# Autodesk Inventor assembly: Shrinkwrap Clamp
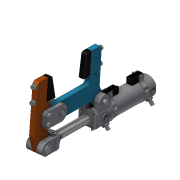
[picture p0: Inventor's stored thumbnail of the model, 180x180]
Saved by Autodesk Inventor 2020.1 (Build 241239000, 239)
## iProperties
Created: 2019-08-27
Part Number: Shrinkwrap Clamp
Document SubType Name: Assembly
Designer: thom_tremblay
Author: thom_tremblay
## Documents named in this file (5)
- C:\Users\thomastremblay\Desktop\Inventor ACP Data\Shrinkwrap Clamp.iam
- C:\Users\thomastremblay\Desktop\Inventor ACP Data\Assemblies\210-103c.iam
- C:\Users\thomastremblay\Desktop\Inventor ACP Data\Assemblies\210-110c.IAM
- C:\Users\thomastremblay\Desktop\Inventor ACP Data\Assemblies\PH-000-002.iam
- C:\Users\thomastremblay\Desktop\Inventor ACP Data\Assemblies\PH-000-001.iam
## Components (4 placed, 4 different names)
1. 210-103c:1 [sub-assembly]
2. 210-110c:1 [sub-assembly]
3. PH-000-002:1 [sub-assembly] — Insert:4
4. PH-000-001:1 [sub-assembly] — Insert:4
## Relationships (6: Insert 4, Mate 2)
- [Insert]: 210-103c:1 ↔ 210-110c:1
- [Insert]: 210-103c:1 ↔ PH-000-001:1
- [Mate]: 210-110c:1 ↔ PH-000-002:1
- [Insert]: 210-103c:1 ↔ PH-000-001:1
- [Mate]: PH-000-002:1 ↔ PH-000-001:1
- Insert:4 (96.52 mm): PH-000-002:1 ↔ PH-000-001:1
